# Autodesk Inventor assembly: PushSwitchAssembly
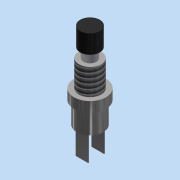
[picture p0: Inventor's stored thumbnail of the model, 180x180]
Saved by Autodesk Inventor 2017 (Build 210142000, 142)
## iProperties
Created: 2016-12-03
Part Number: PushSwitchAssembly
Document SubType Name: Assembly
Designer: techn
Author: techn
## Documents named in this file (4)
- D:\OneDrive\Documents\Other Projects\Submarine\CAD\common\Switches\PushSwitch\PushSwitchAssembly.iam
- D:\OneDrive\Documents\Other Projects\Submarine\CAD\common\Switches\PushSwitch\PushCover.ipt
- D:\OneDrive\Documents\Other Projects\Submarine\CAD\common\Switches\PushSwitch\PushSwitchBody.ipt
- D:\OneDrive\Documents\Other Projects\Submarine\CAD\common\Switches\PushSwitch\PushSwitchRod.ipt
## Components (3 placed, 3 different names)
1. PushCover:1 — Mate:3, Mate:4
2. PushSwitchBody:1 — Mate:1, Mate:2
3. PushSwitchRod:1 — Mate:1, Mate:2, Mate:3, Mate:4
## Relationships (4: Mate 4)
- Mate:1: PushSwitchBody:1 ↔ PushSwitchRod:1
- Mate:2: PushSwitchBody:1 ↔ PushSwitchRod:1
- Mate:3: PushCover:1 ↔ PushSwitchRod:1
- Mate:4: PushCover:1 ↔ PushSwitchRod:1
